# Autodesk Inventor assembly: reaction wheel Assembly
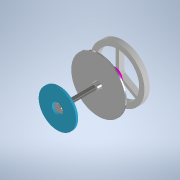
[picture p0: Inventor's stored thumbnail of the model, 180x180]
Saved by Autodesk Inventor 2021 (Build 250183000, 183)
## iProperties
Created: 2021-07-29
Part Number: reaction wheel Assembly
Document SubType Name: Assembly
Designer: samlo
Author: samlo
## Documents named in this file (6)
- C:\Users\samlo\Documents\reaction-wheel\CAD\TEST BENCH\Assembly.iam
- C:\Users\samlo\Documents\reaction-wheel\CAD\TEST BENCH\base.ipt
- C:\Users\samlo\Documents\reaction-wheel\CAD\TEST BENCH\rod and bearing.ipt
- C:\Users\samlo\Documents\reaction-wheel\CAD\TEST BENCH\motor platform.ipt
- C:\Users\samlo\Documents\reaction-wheel\CAD\TEST BENCH\motor.ipt
- C:\Users\samlo\Documents\reaction-wheel\CAD\TEST BENCH\reaction wheel.ipt
## Components (5 placed, 5 different names)
1. base:1 — Rotational:1
2. rod and bearing:1 — Rotational:1, Rigid:1
3. motor platform:1 — Rigid:1, Rigid:2
4. motor:1 — Rigid:2, Rotational:2
5. reaction wheel:1 — Rotational:2
## Relationships (4: RevoluteJoint 2, WeldJoint 2)
- Rotational:1 [RevoluteJoint]: base:1 ↔ rod and bearing:1
- Rigid:1 [WeldJoint]: rod and bearing:1 ↔ motor platform:1
- Rigid:2 [WeldJoint]: motor platform:1 ↔ motor:1
- Rotational:2 [RevoluteJoint] (-9 mm): motor:1 ↔ reaction wheel:1
